# Autodesk Inventor assembly: Zespół1
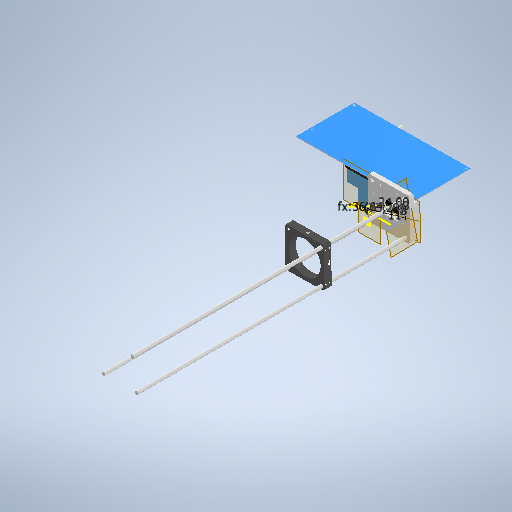
[picture p0: Inventor's stored thumbnail of the model, 512x512]
Saved by Autodesk Inventor 2025.1 (Build 291241000, 241)
## iProperties
Created: 2024-10-25
Part Number: Zespół1
Document SubType Name: Assembly
Designer: PC
Author: PC
## Documents named in this file (6)
- C:\Users\PC\Desktop\fotolito_czesci\nowe\main.iam
- C:\Users\PC\Desktop\fotolito_czesci\nowe\plyta_dmd.iam
- dmd_assembly.iam
- C:\Users\PC\Desktop\fotolito_czesci\rod.ipt
- C:\Users\PC\Desktop\fotolito_czesci\LCP09-Solidworks.ipt
- C:\Users\PC\Desktop\fotolito_czesci\nowe\wyliczenia.ipt
## Components (6 placed, 4 different names)
1. dmd_assembly:1 [sub-assembly] — Zestawiające:2, Zestawiające:3, Zestawiające:4, Zestawiające:5, Zestawiające:6, Równoległe:2, Kątowe:1, Zestawiające:8, Zestawiające:9
2. rod:2 — Zestawiające:2, Zestawiające:6, Zestawiające:10
3. rod:3 — Zestawiające:3, Zestawiające:5
4. rod:4 — Zestawiające:4, Równoległe:2
5. LCP09-Solidworks:1 — Kątowe:1, Zestawiające:10
6. wyliczenia:1 — Zestawiające:8, Zestawiające:9, Zestawiające:11, Kątowe:2
## Relationships (12: Mate 9, Angle 2, Flush 1)
- Zestawiające:2 [Mate]: dmd_assembly:1 ↔ rod:2
- Zestawiające:3 [Mate]: dmd_assembly:1 ↔ rod:3
- Zestawiające:4 [Mate]: dmd_assembly:1 ↔ rod:4
- Zestawiające:5 [Mate]: dmd_assembly:1 ↔ rod:3
- Zestawiające:6 [Mate]: dmd_assembly:1 ↔ rod:2
- Równoległe:2 [Flush]: dmd_assembly:1 ↔ rod:4
- Kątowe:1 [Angle] (0 deg): dmd_assembly:1 ↔ LCP09-Solidworks:1
- Zestawiające:8 [Mate]: dmd_assembly:1 ↔ wyliczenia:1
- Zestawiające:9 [Mate]: dmd_assembly:1 ↔ wyliczenia:1
- Zestawiające:10 [Mate]: rod:2 ↔ LCP09-Solidworks:1
- Zestawiające:11 [Mate]: wyliczenia:1
- Kątowe:2 [Angle] (0 deg): wyliczenia:1
